# Autodesk Inventor assembly: mousetrap19
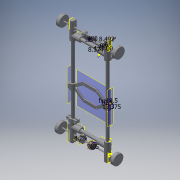
[picture p0: Inventor's stored thumbnail of the model, 180x180]
Saved by Autodesk Inventor 2018 (Build 220112000, 112)
## iProperties
Created: 2018-11-24
Part Number: mousetrap19
Document SubType Name: Assembly
Designer: Prakash
Author: Prakash
## Documents named in this file (17)
- C:\Users\Payal Jindal\Documents\Mousetrap18-19\mousetrap19.iam
- C:\Users\Payal Jindal\Documents\Mousetrap18-19\LBChassis.ipt
- C:\Users\Payal Jindal\Documents\Mousetrap18-19\LFChassis.ipt
- C:\Users\Payal Jindal\Documents\Mousetrap18-19\RBChassiss.ipt
- C:\Users\Payal Jindal\Documents\Mousetrap18-19\RFChassis.ipt
- C:\Users\Payal Jindal\Documents\Mousetrap18-19\LongCF.ipt
- C:\Users\Payal Jindal\Documents\Mousetrap18-19\ShortCF.ipt
- C:\Users\Payal Jindal\Documents\Mousetrap18-19\Axles.ipt
- C:\Users\Payal Jindal\Documents\Mousetrap18-19\93355A310_LOW-STRENGTH STL HEX CPLG NUT.ipt
- C:\Users\Payal Jindal\Documents\Mousetrap18-19\wingnut.ipt
- C:\Users\Payal Jindal\Documents\Mousetrap18-19\springStub.ipt
- C:\Users\Payal Jindal\Documents\Mousetrap18-19\9434K152_MUSIC WIRE PRECISION COMPRESSION SPRING.ipt
- C:\Users\Payal Jindal\Documents\Mousetrap18-19\mousetrapMount.ipt
- C:\Users\Payal Jindal\Documents\Mousetrap18-19\wheels.ipt
- C:\Users\Payal Jindal\Documents\Mousetrap18-19\clampCap.ipt
- C:\Users\Payal Jindal\Documents\Mousetrap18-19\movingSpindle.ipt
- C:\Users\Payal Jindal\Documents\Mousetrap18-19\stationarySpindle.ipt
## Components (23 placed, 16 different names)
1. LBChassis:1 — Mate:1, Mate:2, Mate:11, Mate:15
2. LFChassis:1 — Mate:3, Mate:4, Mate:9, Mate:35, Mate:36
3. RBChassiss:1 — Mate:5, Mate:8, Mate:12, Mate:13, Mate:17, Mate:33, Angle:3
4. RFChassis:1 — Mate:6, Mate:7, Mate:10, Mate:14, Mate:16
5. LongCF:1 — Mate:5, Mate:6, Mate:7, Mate:8, Mate:25, Mate:32
6. LongCF:2 — Mate:1, Mate:2, Mate:3, Mate:4
7. ShortCF:1 — Mate:11, Mate:12, Mate:13, Mate:15
8. ShortCF:2 — Mate:9, Mate:10, Mate:14, Tangent:1
9. Axles:1 — Mate:16, Mate:20, Mate:28, Mate:29, Mate:30, Flush:2, Mate:34
10. Axles:2 — Mate:17, Mate:26, Mate:27, Flush:3, Mate:31, Mate:40, Mate:41
11. 93355A310_LOW-STRENGTH STL HEX CPLG NUT:1 — Mate:20, Angle:4, Flush:4
12. wingnut:1 — Mate:34, Angle:4, Flush:4, Tangent:1
13. mousetrapMount:1 — Mate:25, Angle:2
14. wheels:1 — Mate:26, Mate:27
15. wheels:2 — Mate:30, Flush:2
16. wheels:3 — Flush:3, Mate:31
17. wheels:4 — Mate:28, Mate:29
18. clampCap:1 — Mate:32, Mate:33, Angle:3
19. 9434K152_MUSIC WIRE PRECISION COMPRESSION SPRING:1 — Mate:37, Mate:38
20. springStub:1 — Mate:35, Mate:36, Mate:37, Mate:38
21. 93355A310_LOW-STRENGTH STL HEX CPLG NUT:2 — Mate:39, Angle:5, Flush:5
22. movingSpindle:1 — Mate:39, Angle:5, Flush:5, Mate:41
23. stationarySpindle:1 — Mate:40
## Relationships (44: Mate 35, Angle 4, Flush 4, Tangent 1)
- Mate:1: LBChassis:1 ↔ LongCF:2
- Mate:2: LBChassis:1 ↔ LongCF:2
- Mate:3: LFChassis:1 ↔ LongCF:2
- Mate:4: LFChassis:1 ↔ LongCF:2
- Mate:5: RBChassiss:1 ↔ LongCF:1
- Mate:6: RFChassis:1 ↔ LongCF:1
- Mate:7: RFChassis:1 ↔ LongCF:1
- Mate:8: RBChassiss:1 ↔ LongCF:1
- Mate:9: LFChassis:1 ↔ ShortCF:2
- Mate:10: RFChassis:1 ↔ ShortCF:2
- Mate:11: LBChassis:1 ↔ ShortCF:1
- Mate:12: RBChassiss:1 ↔ ShortCF:1
- Mate:13: RBChassiss:1 ↔ ShortCF:1
- Mate:14: RFChassis:1 ↔ ShortCF:2
- Mate:15: LBChassis:1 ↔ ShortCF:1
- Mate:16: RFChassis:1 ↔ Axles:1
- Mate:17: RBChassiss:1 ↔ Axles:2
- Mate:20: Axles:1 ↔ 93355A310_LOW-STRENGTH STL HEX CPLG NUT:1
- Mate:25: LongCF:1 ↔ mousetrapMount:1
- Angle:2 (0 deg): mousetrapMount:1
- Mate:26: Axles:2 ↔ wheels:1
- Mate:27: Axles:2 ↔ wheels:1
- Mate:28: Axles:1 ↔ wheels:4
- Mate:29: Axles:1 ↔ wheels:4
- Mate:30: Axles:1 ↔ wheels:2
- Flush:2: Axles:1 ↔ wheels:2
- Flush:3: Axles:2 ↔ wheels:3
- Mate:31: Axles:2 ↔ wheels:3
- Mate:32: LongCF:1 ↔ clampCap:1
- Mate:33: RBChassiss:1 ↔ clampCap:1
- Angle:3 (0 deg): RBChassiss:1 ↔ clampCap:1
- Mate:34: Axles:1 ↔ wingnut:1
- Angle:4 (0 deg): 93355A310_LOW-STRENGTH STL HEX CPLG NUT:1 ↔ wingnut:1
- Flush:4: 93355A310_LOW-STRENGTH STL HEX CPLG NUT:1 ↔ wingnut:1
- Tangent:1: ShortCF:2 ↔ wingnut:1
- Mate:35: LFChassis:1 ↔ springStub:1
- Mate:36: LFChassis:1 ↔ springStub:1
- Mate:37: 9434K152_MUSIC WIRE PRECISION COMPRESSION SPRING:1 ↔ springStub:1
- Mate:38: 9434K152_MUSIC WIRE PRECISION COMPRESSION SPRING:1 ↔ springStub:1
- Mate:39: 93355A310_LOW-STRENGTH STL HEX CPLG NUT:2 ↔ movingSpindle:1
- Angle:5 (0 deg): 93355A310_LOW-STRENGTH STL HEX CPLG NUT:2 ↔ movingSpindle:1
- Flush:5: 93355A310_LOW-STRENGTH STL HEX CPLG NUT:2 ↔ movingSpindle:1
- Mate:40: Axles:2 ↔ stationarySpindle:1
- Mate:41: Axles:2 ↔ movingSpindle:1
